# Autodesk Inventor assembly: steering_queens_pair
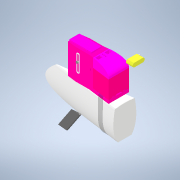
[picture p0: Inventor's stored thumbnail of the model, 180x180]
Saved by Autodesk Inventor 2020 (Build 240168000, 168)
## iProperties
Created: 2019-09-18
Part Number: steering_queens_pair
Document SubType Name: Assembly
Designer: suchanek
Author: suchanek
## Documents named in this file (15)
- D:\suchanek\programming\rowing_steering\model_final\steering_queens_pair.iam
- D:\suchanek\programming\rowing_steering\model_final\boat_pair_queens.ipt
- D:\suchanek\programming\rowing_steering\model_final\rudder_pair_queens.ipt
- D:\suchanek\programming\rowing_steering\model_final\hull_main.ipt
- D:\suchanek\programming\rowing_steering\model_final\hull_servo.ipt
- D:\suchanek\programming\rowing_steering\model_final\servo.ipt
- D:\suchanek\programming\rowing_steering\model_final\servo_bit.ipt
- D:\suchanek\programming\rowing_steering\model_final\Strap.ipt
- D:\suchanek\programming\rowing_steering\model_final\hull_electronics.ipt
- D:\suchanek\programming\rowing_steering\model_final\hull_electronics_top.ipt
- D:\suchanek\programming\rowing_steering\model_final\arduino.iam
- D:\suchanek\programming\rowing_steering\model_final\battery.ipt
- D:\suchanek\programming\rowing_steering\model_final\battery_small.ipt
- D:\suchanek\programming\rowing_steering\model_final\hull_rudder_tube_clamp.ipt
- D:\suchanek\Documents\Inventor\Content Center Files\R2020\en-US\AS 1110\AS 1110 - M6 x 20.ipt
## Components (17 placed, 14 different names)
1. boat_pair_queens:1 — Rotational:1, Cylindrical:1, Angle:1, Tangent:1, Mate:7, Tangent:4
2. rudder_pair_queens:1 — Rotational:1, Angle:3
3. hull_main:1 — Cylindrical:1, Angle:1, Tangent:1, Cylindrical:2, Angle:2, Mate:3, Mate:4, Flush:1, Flush:2, Cylindrical:5, Mate:8, Cylindrical:6, Mate:16
4. hull_servo:1 — Rotational:2, Mate:1, Cylindrical:2, Angle:2, Cylindrical:3, Cylindrical:4
5. servo:1 — Rotational:2, Mate:1, Rotational:3
6. servo_bit:1 — Angle:3, Rotational:3, Mate:7
7. AS 1110 - Metric M6 x 20:1 — Cylindrical:3, Mate:3
8. AS 1110 - Metric M6 x 20:2 — Cylindrical:4, Mate:4
9. Strap:1 — Flush:1, Flush:2
10. hull_electronics:1 — Cylindrical:5, Mate:8, Flush:3, Rotational:4, Flush:4, Angle:5, Angle:6, Mate:14, Mate:15, Flush:6, Mate:17
11. hull_electronics_top:1 — Flush:3, Rotational:4, Flush:4
12. arduino:1 [sub-assembly] — Mate:14, Mate:15, Flush:6
13. battery:1 — Rigid:1, Rigid:2
14. battery:2 — Rigid:1
15. battery:5 — Rigid:2, Mate:17
16. battery_small:1 — Angle:5, Angle:6
17. hull_rudder_tube_clamp:1 — Cylindrical:6, Mate:16, Tangent:4
## Relationships (33: Mate 9, CylindricalJoint 6, Angle 5, Flush 5, RevoluteJoint 4, Tangent 2, WeldJoint 2)
- Rotational:1 [RevoluteJoint]: boat_pair_queens:1 ↔ rudder_pair_queens:1
- Cylindrical:1: boat_pair_queens:1 ↔ hull_main:1
- Angle:1 (0 deg): boat_pair_queens:1 ↔ hull_main:1
- Tangent:1: boat_pair_queens:1 ↔ hull_main:1
- Rotational:2 [RevoluteJoint]: hull_servo:1 ↔ servo:1
- Mate:1: hull_servo:1 ↔ servo:1
- Cylindrical:2: hull_main:1 ↔ hull_servo:1
- Angle:2 (0 deg): hull_main:1 ↔ hull_servo:1
- Angle:3 (0 deg): rudder_pair_queens:1 ↔ servo_bit:1
- Cylindrical:3: hull_servo:1 ↔ AS 1110 - Metric M6 x 20:1
- Cylindrical:4: hull_servo:1 ↔ AS 1110 - Metric M6 x 20:2
- Mate:3 (1 mm): hull_main:1 ↔ AS 1110 - Metric M6 x 20:1
- Mate:4 (1 mm): hull_main:1 ↔ AS 1110 - Metric M6 x 20:2
- Flush:1: hull_main:1 ↔ Strap:1
- Flush:2 (20 mm): hull_main:1 ↔ Strap:1
- Rotational:3 [RevoluteJoint]: servo:1 ↔ servo_bit:1
- Mate:7: boat_pair_queens:1 ↔ servo_bit:1
- Cylindrical:5: hull_main:1 ↔ hull_electronics:1
- Mate:8: hull_main:1 ↔ hull_electronics:1
- Flush:3: hull_electronics:1 ↔ hull_electronics_top:1
- Rotational:4 [RevoluteJoint]: hull_electronics:1 ↔ hull_electronics_top:1
- Flush:4: hull_electronics:1 ↔ hull_electronics_top:1
- Rigid:1 [WeldJoint]: battery:1 ↔ battery:2
- Angle:5 (0 deg): hull_electronics:1 ↔ battery_small:1
- Angle:6 (0 deg): hull_electronics:1 ↔ battery_small:1
- Mate:14: hull_electronics:1 ↔ arduino:1
- Mate:15: hull_electronics:1 ↔ arduino:1
- Flush:6: hull_electronics:1 ↔ arduino:1
- Cylindrical:6: hull_main:1 ↔ hull_rudder_tube_clamp:1
- Mate:16: hull_main:1 ↔ hull_rudder_tube_clamp:1
- Tangent:4: boat_pair_queens:1 ↔ hull_rudder_tube_clamp:1
- Rigid:2 [WeldJoint]: battery:1 ↔ battery:5
- Mate:17: hull_electronics:1 ↔ battery:5
